# Autodesk Inventor assembly: Assembly2
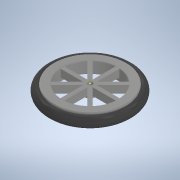
[picture p0: Inventor's stored thumbnail of the model, 180x180]
Saved by Autodesk Inventor 2021 (Build 250183000, 183)
## iProperties
Created: 2021-03-19
Part Number: Assembly2
Document SubType Name: Assembly
Designer: uriel
Author: uriel
## Documents named in this file (3)
- C:\Users\uriel\Documents\Escuela\LABORATORIO DISEÑO Y MANUFACTURA ASISTIDA POR COMPUTADORA\Practica 2\Assembly2.iam
- C:\Users\uriel\Documents\Inventor\CuerpoLlanta.ipt
- C:\Users\uriel\Documents\Escuela\LABORATORIO DISEÑO Y MANUFACTURA ASISTIDA POR COMPUTADORA\Practica 2\Imported Components\Llanta\Llanta.ipt
## Components (2 placed, 2 different names)
1. CuerpoLlanta:1 — Mate:1, Flush:1, Flush:2
2. Llanta:1 — Mate:1
## Relationships (3: Flush 2, Mate 1)
- Mate:1: CuerpoLlanta:1 ↔ Llanta:1
- Flush:1: CuerpoLlanta:1
- Flush:2: CuerpoLlanta:1
